# Autodesk Inventor assembly: V0.2R1 Tulip Mod master v35
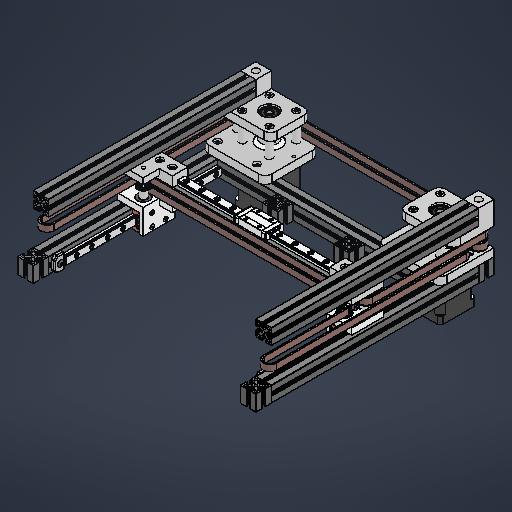
[picture p0: Inventor's stored thumbnail of the model, 512x512]
Saved by Autodesk Inventor 2026 (Build 300175050, 175E)
## iProperties
Created: 2025-05-23
Part Number: V0.2R1 Tulip Mod master v35
Document SubType Name: Assembly
Designer: Joshua Eah
Sending System: Autodesk Translation Framework v13.20.0.188
Preprocessor: ST-DEVELOPER v20
Title: V0.2R1 Tulip Mod master v35.step
## Documents named in this file (10)
- C:\Users\Joshua Eah\Documents\GitHub\Voron-0\CAD\Tulip - Machined Parts\Tulip Mod Master\Master Assembly.iam
- C:\Users\Joshua Eah\Documents\GitHub\Voron-0\CAD\Tulip - Machined Parts\Tulip Mod Master\Frame.iam
- C:\Users\Joshua Eah\Documents\GitHub\Voron-0\CAD\Tulip - Machined Parts\AB Drives\A Drive\A_Drive.iam
- C:\Users\Joshua Eah\Documents\GitHub\Voron-0\CAD\Tulip - Machined Parts\AB Drives\B Drive\B_Drive.iam
- C:\Users\Joshua Eah\Documents\GitHub\Voron-0\CAD\Tulip - Machined Parts\Tulip Mod Master\MGN7 Rail 150mm (1).iam
- C:\Users\Joshua Eah\Documents\GitHub\Voron-0\CAD\Tulip - Machined Parts\Tulip Mod Master\MGN7 Rail 150mm (2).iam
- C:\Users\Joshua Eah\Documents\GitHub\Voron-0\CAD\Tulip - Machined Parts\Tulip Mod Master\MGN7H Carriage (1).ipt
- C:\Users\Joshua Eah\Documents\GitHub\Voron-0\CAD\Tulip - Machined Parts\Tulip Mod Master\MGN7H Carriage (2).ipt
- C:\Users\Joshua Eah\Documents\GitHub\Voron-0\CAD\Tulip - Machined Parts\Tulip Mod Master\Belts.iam
- C:\Users\Joshua Eah\Documents\GitHub\Voron-0\CAD\Tulip - Machined Parts\Tulip Mod Master\X Axis.iam
## Components (9 placed, 9 different names)
1. Frame:1 [sub-assembly] — Insert:1, Angle:1, Angle:2, Angle:3, Flush:1, Flush:2, Mate:2, Mate:3, Mate:4, Mate:5, Insert:7
2. X Axis:1 [sub-assembly] — Insert:5, Insert:6, Transitional:1
3. A_Drive:1 [sub-assembly] — Insert:7
4. B_Drive:1 [sub-assembly] — Insert:1, Angle:1
5. MGN7 Rail 150mm (1):1 [sub-assembly] — Cylindrical:4, Cylindrical:2, Angle:2, Flush:2, Mate:2, Mate:5
6. MGN7 Rail 150mm (2):1 [sub-assembly] — Cylindrical:1, Cylindrical:3, Angle:3, Flush:1, Mate:3, Mate:4
7. MGN7H Carriage (1):1 — Cylindrical:4, Cylindrical:2, Insert:5
8. MGN7H Carriage (2):1 — Cylindrical:1, Cylindrical:3, Insert:6
9. Belts:1 [sub-assembly] — Transitional:1
## Relationships (18: Insert 4, CylindricalJoint 4, Mate 4, Angle 3, Flush 2, Transitional 1)
- Insert:1: Frame:1 ↔ B_Drive:1
- Angle:1 (0 deg): Frame:1 ↔ B_Drive:1
- Cylindrical:1: MGN7 Rail 150mm (2):1 ↔ MGN7H Carriage (2):1
- Cylindrical:4: MGN7 Rail 150mm (1):1 ↔ MGN7H Carriage (1):1
- Cylindrical:2: MGN7 Rail 150mm (1):1 ↔ MGN7H Carriage (1):1
- Cylindrical:3: MGN7 Rail 150mm (2):1 ↔ MGN7H Carriage (2):1
- Insert:5: X Axis:1 ↔ MGN7H Carriage (1):1
- Angle:2 (0 deg): Frame:1 ↔ MGN7 Rail 150mm (1):1
- Angle:3 (0 deg): Frame:1 ↔ MGN7 Rail 150mm (2):1
- Flush:1 (4 mm): Frame:1 ↔ MGN7 Rail 150mm (2):1
- Flush:2 (4 mm): Frame:1 ↔ MGN7 Rail 150mm (1):1
- Mate:2: Frame:1 ↔ MGN7 Rail 150mm (1):1
- Mate:3: Frame:1 ↔ MGN7 Rail 150mm (2):1
- Mate:4: Frame:1 ↔ MGN7 Rail 150mm (2):1
- Mate:5: Frame:1 ↔ MGN7 Rail 150mm (1):1
- Insert:6: X Axis:1 ↔ MGN7H Carriage (2):1
- Transitional:1: X Axis:1 ↔ Belts:1
- Insert:7: Frame:1 ↔ A_Drive:1
